# Autodesk Inventor assembly: ELEV_000_FULLASMBLY
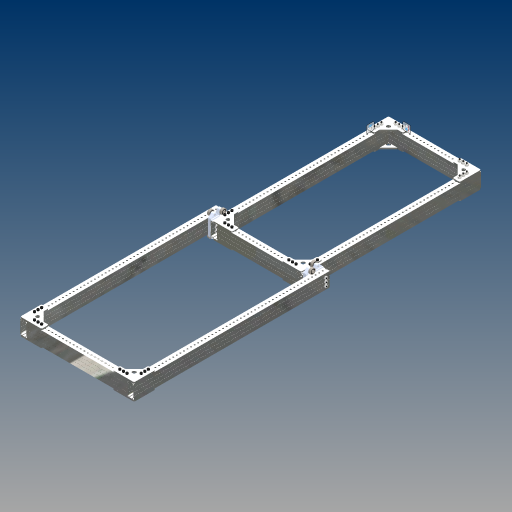
[picture p0: Inventor's stored thumbnail of the model, 512x512]
Saved by Autodesk Inventor 2024.3 (Build 283343000, 343)
## iProperties
Created: 2024-11-25
Part Number: ELEV_000_FULLASMBLY
Document SubType Name: Assembly
Designer: Kenji
Mass: 3407.89 g
Surface Area: 12378 cm^2
Volume: 1206.36 cm^3
Density: 2.82493 g/cm^3
Author: Kenji
## Documents named in this file (22)
- C:\Users\Kenji\Documents\GitHub\1622-2024-Casino-Clash-CAD-A-Thon\Elevator\ELEV_000_FULLASMBLY.iam
- C:\Users\Kenji\Documents\GitHub\1622-2024-Casino-Clash-CAD-A-Thon\Elevator\ELEV_001_BAR1(27.500 in).ipt
- C:\Users\Kenji\Documents\GitHub\1622-2024-Casino-Clash-CAD-A-Thon\Elevator\ELEV_002_BAR2(14.000 in).ipt
- C:\Users\Kenji\Documents\GitHub\1622-2024-Casino-Clash-CAD-A-Thon\Elevator\ELEV_003_BAR3(25.000 in).ipt
- C:\Users\Kenji\Documents\GitHub\1622-2024-Casino-Clash-CAD-A-Thon\COTS Library\Motion\BearingBlocks\ElevatorBlocks\WCP-0897_InlineBearingBlock.iam
- C:\Users\Kenji\Documents\GitHub\1622-2024-Casino-Clash-CAD-A-Thon\Elevator\ELEV_004_BAR4(12.000 in).ipt
- C:\Users\Kenji\Documents\GitHub\1622-2024-Casino-Clash-CAD-A-Thon\Elevator\ELEV_005_SUPBRK1.ipt
- C:\Users\Kenji\Documents\GitHub\1622-2024-Casino-Clash-CAD-A-Thon\COTS Library\Fasteners\Nuts\COTS_90633A411_Low-Strength Steel Thin Nylon-Insert Locknut_10-32.ipt
- C:\Users\Kenji\Documents\GitHub\1622-2024-Casino-Clash-CAD-A-Thon\Elevator\ELEV_006_SUPBRK1_THRD.ipt
- C:\Users\Kenji\Documents\GitHub\1622-2024-Casino-Clash-CAD-A-Thon\COTS Library\Fasteners\Bolts\Socket-Head\10-32\COTS_90044A121_Black-Oxide Alloy Steel Socket Head Screw_10-32_2.5in.ipt
- C:\Users\Kenji\Documents\GitHub\1622-2024-Casino-Clash-CAD-A-Thon\COTS Library\Fasteners\Bolts\Socket-Head\10-32\COTS_90044A202_Black-Oxide Alloy Steel Socket Head Screw_1-.375.ipt
- C:\Users\Kenji\Documents\GitHub\1622-2024-Casino-Clash-CAD-A-Thon\COTS Library\Fasteners\Bolts\Socket-Head\10-32\COTS_91251A342_Black-Oxide Alloy Steel Socket Head Screw_.5in.ipt
- C:\Users\Kenji\Documents\GitHub\1622-2024-Casino-Clash-CAD-A-Thon\Elevator\ELEV_007_SUPBRK2.ipt
- C:\Users\Kenji\Documents\GitHub\1622-2024-Casino-Clash-CAD-A-Thon\COTS Library\Fasteners\Bolts\Socket-Head\10-32\COTS_91251A359_Black-Oxide Alloy Steel Socket Head Screw_10-32_2_3-4in.ipt
- C:\Users\Kenji\Documents\GitHub\1622-2024-Casino-Clash-CAD-A-Thon\COTS Library\Fasteners\Nuts\COTS_90631A411_Low-Strength Steel Nylon-Insert Locknut_10-32.ipt
- C:\Users\Kenji\Documents\GitHub\1622-2024-Casino-Clash-CAD-A-Thon\Elevator\ELEV_008_SUPBRK3.ipt
- C:\Users\Kenji\Documents\GitHub\1622-2024-Casino-Clash-CAD-A-Thon\Elevator\ELEV_000_FULLASMBLY\AIP\FEA\ew6g7bhkw.fins
- C:\Users\Kenji\Documents\GitHub\1622-2024-Casino-Clash-CAD-A-Thon\Elevator\ELEV_000_FULLASMBLY\AIP\FEA\ew6g7bhkw.fsat
- C:\Users\Kenji\Documents\GitHub\1622-2024-Casino-Clash-CAD-A-Thon\Elevator\ELEV_000_FULLASMBLY\AIP\FEA\ew6g7bhkw.ftes
- C:\Users\Kenji\Documents\GitHub\1622-2024-Casino-Clash-CAD-A-Thon\Elevator\ELEV_000_FULLASMBLY\AIP\FEA\ew6g7bhkw.fwiz
- C:\Users\Kenji\Documents\GitHub\1622-2024-Casino-Clash-CAD-A-Thon\Elevator\ELEV_000_FULLASMBLY\AIP\FEA\ew6g7biao.fmsh
- C:\Users\Kenji\Documents\GitHub\1622-2024-Casino-Clash-CAD-A-Thon\Elevator\ELEV_000_FULLASMBLY\AIP\FEA\ew6g7bibk.fres
## Components (107 placed, 15 different names)
1. ELEV_001_BAR1(27.500 in):1 — Flush:1, Flush:2, Mate:1, Mate:2, Flush:7, Tangent:2, Mate:10, Flush:11, Mate:11, Mate:78, Mate:133, Mate:136, Mate:137
2. ELEV_001_BAR1(27.500 in):2 — Flush:1, Flush:2, Mate:1, Flush:3, Flush:4, Mate:3, Angle:1, Mate:4, Flush:8, Angle:2, Mate:74, Mate:128, Mate:131
3. ELEV_002_BAR2(14.000 in):1 — Flush:3, Flush:4, Mate:2, Mate:127, Flush:24, Mate:132, Mate:134, Mate:135
4. ELEV_003_BAR3(25.000 in):1 — Flush:5, Flush:6, Flush:7, Mate:8, Flush:10, Mate:9, Mate:82, Flush:19, Flush:21
5. ELEV_003_BAR3(25.000 in):2 — Flush:5, Flush:6, Tangent:1, Angle:2, Mate:5, Angle:3, Mate:6, Flush:9, Mate:12, Flush:12, Flush:13, Mate:13, Flush:14, Mate:14, Mate:16, Mate:62, Mate:86, Flush:17, Flush:22
6. WCP-0897_InlineBearingBlock:1 [sub-assembly] — Mate:5, Angle:3, Mate:6, Flush:9, Mate:83, Mate:84
7. WCP-0897_InlineBearingBlock:2 [sub-assembly] — Mate:3, Angle:1, Mate:4, Tangent:1, Flush:8, Mate:71, Mate:72
8. WCP-0897_InlineBearingBlock:3 [sub-assembly] — Mate:8, Flush:10, Mate:9, Tangent:2, Mate:37, Mate:79, Mate:80
9. WCP-0897_InlineBearingBlock:4 [sub-assembly] — Mate:10, Flush:11, Mate:11, Mate:37, Mate:75, Mate:76
10. ELEV_004_BAR4(12.000 in):1 — Mate:12, Flush:12, Flush:13, Mate:17, Mate:18, Mate:19, Angle:4, Mate:20, Mate:42, Mate:45, Mate:60, Flush:15, Mate:61
11. ELEV_004_BAR4(12.000 in):2 — Mate:13, Flush:14, Mate:14, Flush:16, Flush:18, Mate:88, Flush:20, Mate:89, Flush:23, Mate:90, Mate:110
12. ELEV_005_SUPBRK1:1 — Mate:16, Mate:17, Mate:18, Mate:67, Mate:68, Mate:69, Mate:70
13. ELEV_005_SUPBRK1:2 — Mate:19, Angle:4, Mate:20, Mate:63, Mate:64, Mate:65, Mate:66
14. ELEV_006_SUPBRK1_THRD:1 — Mate:42, Mate:61, Mate:62
15. ELEV_006_SUPBRK1_THRD:2 — Mate:45, Mate:60, Flush:15
16. ELEV_007_SUPBRK2:1 — Flush:16, Flush:17, Mate:110, Mate:120, Mate:122
17. ELEV_007_SUPBRK2:2 — Flush:18, Flush:19, Mate:88, Mate:124, Mate:126
18. ELEV_007_SUPBRK2:3 — Flush:22, Flush:23, Mate:90, Mate:115, Mate:116, Mate:117, Mate:118
19. ELEV_007_SUPBRK2:4 — Flush:20, Flush:21, Mate:89, Mate:111, Mate:112, Mate:113, Mate:114
20. ELEV_008_SUPBRK3:1 — Mate:127, Flush:24, Mate:128, Mate:129, Mate:130, Mate:138, Mate:139, Mate:144, Mate:145
21. ELEV_008_SUPBRK3:2 — Mate:129, Mate:130, Mate:131, Mate:148, Mate:149
22. ELEV_008_SUPBRK3:3 — Mate:132, Mate:133, Mate:134, Mate:151, Mate:153
23. ELEV_008_SUPBRK3:4 — Mate:135, Mate:136, Mate:137, Mate:140, Mate:141, Mate:142, Mate:143
24. COTS_90044A121_Black-Oxide Alloy Steel Socket Head Screw_10-32_2.5in:1 — Mate:63, Mate:64
25. COTS_90044A121_Black-Oxide Alloy Steel Socket Head Screw_10-32_2.5in:5
26. COTS_90044A121_Black-Oxide Alloy Steel Socket Head Screw_10-32_2.5in:6
27. COTS_90044A121_Black-Oxide Alloy Steel Socket Head Screw_10-32_2.5in:4 — Mate:65, Mate:66
28. COTS_90044A121_Black-Oxide Alloy Steel Socket Head Screw_10-32_2.5in:7
29. COTS_90044A121_Black-Oxide Alloy Steel Socket Head Screw_10-32_2.5in:8
30. COTS_90044A121_Black-Oxide Alloy Steel Socket Head Screw_10-32_2.5in:3 — Mate:68, Mate:70
31. COTS_90044A121_Black-Oxide Alloy Steel Socket Head Screw_10-32_2.5in:9
32. COTS_90044A121_Black-Oxide Alloy Steel Socket Head Screw_10-32_2.5in:10
33. COTS_90044A121_Black-Oxide Alloy Steel Socket Head Screw_10-32_2.5in:2 — Mate:67, Mate:69
34. COTS_90044A121_Black-Oxide Alloy Steel Socket Head Screw_10-32_2.5in:11
35. COTS_90044A121_Black-Oxide Alloy Steel Socket Head Screw_10-32_2.5in:12
36. COTS_90044A202_Black-Oxide Alloy Steel Socket Head Screw_1-.375:1 — Mate:71, Mate:72, Mate:73
37. COTS_90633A411_Low-Strength Steel Thin Nylon-Insert Locknut_10-32:1 — Mate:73, Mate:74
38. COTS_90044A202_Black-Oxide Alloy Steel Socket Head Screw_1-.375:2
39. COTS_90633A411_Low-Strength Steel Thin Nylon-Insert Locknut_10-32:2
40. COTS_90044A202_Black-Oxide Alloy Steel Socket Head Screw_1-.375:3
41. COTS_90633A411_Low-Strength Steel Thin Nylon-Insert Locknut_10-32:3
42. COTS_90633A411_Low-Strength Steel Thin Nylon-Insert Locknut_10-32:4 — Mate:77, Mate:78
43. COTS_90044A202_Black-Oxide Alloy Steel Socket Head Screw_1-.375:4 — Mate:75, Mate:76, Mate:77
44. COTS_90633A411_Low-Strength Steel Thin Nylon-Insert Locknut_10-32:5
45. COTS_90044A202_Black-Oxide Alloy Steel Socket Head Screw_1-.375:5
46. COTS_90633A411_Low-Strength Steel Thin Nylon-Insert Locknut_10-32:6
47. COTS_90044A202_Black-Oxide Alloy Steel Socket Head Screw_1-.375:6
48. COTS_91251A342_Black-Oxide Alloy Steel Socket Head Screw_.5in:1 — Mate:79, Mate:80, Mate:81
49. COTS_90633A411_Low-Strength Steel Thin Nylon-Insert Locknut_10-32:7 — Mate:81, Mate:82
50. COTS_91251A342_Black-Oxide Alloy Steel Socket Head Screw_.5in:2
51. COTS_90633A411_Low-Strength Steel Thin Nylon-Insert Locknut_10-32:8
52. COTS_91251A342_Black-Oxide Alloy Steel Socket Head Screw_.5in:3
53. COTS_90633A411_Low-Strength Steel Thin Nylon-Insert Locknut_10-32:9
54. COTS_90633A411_Low-Strength Steel Thin Nylon-Insert Locknut_10-32:10 — Mate:85, Mate:86
55. COTS_91251A342_Black-Oxide Alloy Steel Socket Head Screw_.5in:4 — Mate:83, Mate:84, Mate:85
56. COTS_90633A411_Low-Strength Steel Thin Nylon-Insert Locknut_10-32:11
57. COTS_91251A342_Black-Oxide Alloy Steel Socket Head Screw_.5in:5
58. COTS_90633A411_Low-Strength Steel Thin Nylon-Insert Locknut_10-32:12
59. COTS_91251A342_Black-Oxide Alloy Steel Socket Head Screw_.5in:6
60. COTS_91251A359_Black-Oxide Alloy Steel Socket Head Screw_10-32_2_3-4in:3 — Mate:111, Mate:112, Mate:123
61. COTS_90631A411_Low-Strength Steel Nylon-Insert Locknut_10-32:2 — Mate:123, Mate:124
62. COTS_91251A359_Black-Oxide Alloy Steel Socket Head Screw_10-32_2_3-4in:5
63. COTS_90631A411_Low-Strength Steel Nylon-Insert Locknut_10-32:5
64. COTS_91251A359_Black-Oxide Alloy Steel Socket Head Screw_10-32_2_3-4in:6
65. COTS_90631A411_Low-Strength Steel Nylon-Insert Locknut_10-32:6
66. COTS_91251A359_Black-Oxide Alloy Steel Socket Head Screw_10-32_2_3-4in:1 — Mate:113, Mate:114, Mate:125
67. COTS_91251A359_Black-Oxide Alloy Steel Socket Head Screw_10-32_2_3-4in:7
68. COTS_91251A359_Black-Oxide Alloy Steel Socket Head Screw_10-32_2_3-4in:8
69. COTS_91251A359_Black-Oxide Alloy Steel Socket Head Screw_10-32_2_3-4in:2 — Mate:115, Mate:118, Mate:121
70. COTS_90631A411_Low-Strength Steel Nylon-Insert Locknut_10-32:4 — Mate:121, Mate:122
71. COTS_91251A359_Black-Oxide Alloy Steel Socket Head Screw_10-32_2_3-4in:9
72. COTS_90631A411_Low-Strength Steel Nylon-Insert Locknut_10-32:7
73. COTS_91251A359_Black-Oxide Alloy Steel Socket Head Screw_10-32_2_3-4in:10
74. COTS_90631A411_Low-Strength Steel Nylon-Insert Locknut_10-32:8
75. COTS_90631A411_Low-Strength Steel Nylon-Insert Locknut_10-32:3 — Mate:119, Mate:120
76. COTS_91251A359_Black-Oxide Alloy Steel Socket Head Screw_10-32_2_3-4in:4 — Mate:116, Mate:117, Mate:119
77. COTS_90631A411_Low-Strength Steel Nylon-Insert Locknut_10-32:9
78. COTS_91251A359_Black-Oxide Alloy Steel Socket Head Screw_10-32_2_3-4in:11
79. COTS_90631A411_Low-Strength Steel Nylon-Insert Locknut_10-32:10
80. COTS_91251A359_Black-Oxide Alloy Steel Socket Head Screw_10-32_2_3-4in:12
81. COTS_90631A411_Low-Strength Steel Nylon-Insert Locknut_10-32:1 — Mate:125, Mate:126
82. COTS_90631A411_Low-Strength Steel Nylon-Insert Locknut_10-32:11
83. COTS_90631A411_Low-Strength Steel Nylon-Insert Locknut_10-32:12
84. COTS_90631A411_Low-Strength Steel Nylon-Insert Locknut_10-32:14 — Mate:152, Mate:153
85. COTS_91251A359_Black-Oxide Alloy Steel Socket Head Screw_10-32_2_3-4in:14 — Mate:140, Mate:143, Mate:152
86. COTS_90631A411_Low-Strength Steel Nylon-Insert Locknut_10-32:17
87. COTS_91251A359_Black-Oxide Alloy Steel Socket Head Screw_10-32_2_3-4in:17
88. COTS_90631A411_Low-Strength Steel Nylon-Insert Locknut_10-32:18
89. COTS_91251A359_Black-Oxide Alloy Steel Socket Head Screw_10-32_2_3-4in:18
90. COTS_91251A359_Black-Oxide Alloy Steel Socket Head Screw_10-32_2_3-4in:13 — Mate:141, Mate:142, Mate:150
91. COTS_90631A411_Low-Strength Steel Nylon-Insert Locknut_10-32:15 — Mate:150, Mate:151
92. COTS_91251A359_Black-Oxide Alloy Steel Socket Head Screw_10-32_2_3-4in:19
93. COTS_90631A411_Low-Strength Steel Nylon-Insert Locknut_10-32:19
94. COTS_91251A359_Black-Oxide Alloy Steel Socket Head Screw_10-32_2_3-4in:20
95. COTS_90631A411_Low-Strength Steel Nylon-Insert Locknut_10-32:20
96. COTS_91251A359_Black-Oxide Alloy Steel Socket Head Screw_10-32_2_3-4in:15 — Mate:139, Mate:145, Mate:147
97. COTS_90631A411_Low-Strength Steel Nylon-Insert Locknut_10-32:13 — Mate:147, Mate:149
98. COTS_91251A359_Black-Oxide Alloy Steel Socket Head Screw_10-32_2_3-4in:21
99. COTS_90631A411_Low-Strength Steel Nylon-Insert Locknut_10-32:21
100. COTS_91251A359_Black-Oxide Alloy Steel Socket Head Screw_10-32_2_3-4in:22
101. COTS_90631A411_Low-Strength Steel Nylon-Insert Locknut_10-32:22
102. COTS_90631A411_Low-Strength Steel Nylon-Insert Locknut_10-32:16 — Mate:146, Mate:148
103. COTS_91251A359_Black-Oxide Alloy Steel Socket Head Screw_10-32_2_3-4in:16 — Mate:138, Mate:144, Mate:146
104. COTS_90631A411_Low-Strength Steel Nylon-Insert Locknut_10-32:23
105. COTS_91251A359_Black-Oxide Alloy Steel Socket Head Screw_10-32_2_3-4in:23
106. COTS_90631A411_Low-Strength Steel Nylon-Insert Locknut_10-32:24
107. COTS_91251A359_Black-Oxide Alloy Steel Socket Head Screw_10-32_2_3-4in:24
## Component patterns: (3 elements, first: COTS_90044A121_Black-Oxide Alloy Steel Socket Head Screw_10-32_2.5in:1), (3 elements, first: COTS_90044A121_Black-Oxide Alloy Steel Socket Head Screw_10-32_2.5in:4), (3 elements, first: COTS_90044A121_Black-Oxide Alloy Steel Socket Head Screw_10-32_2.5in:3), (3 elements, first: COTS_90044A121_Black-Oxide Alloy Steel Socket Head Screw_10-32_2.5in:2), (3 elements, first: COTS_90044A202_Black-Oxide Alloy Steel Socket Head Screw_1-.375:1 + COTS_90633A411_Low-Strength Steel Thin Nylon-Insert Locknut_10-32:1), (3 elements, first: COTS_90633A411_Low-Strength Steel Thin Nylon-Insert Locknut_10-32:4 + COTS_90044A202_Black-Oxide Alloy Steel Socket Head Screw_1-.375:4), (3 elements, first: COTS_91251A342_Black-Oxide Alloy Steel Socket Head Screw_.5in:1 + COTS_90633A411_Low-Strength Steel Thin Nylon-Insert Locknut_10-32:7), (3 elements, first: COTS_90633A411_Low-Strength Steel Thin Nylon-Insert Locknut_10-32:10 + COTS_91251A342_Black-Oxide Alloy Steel Socket Head Screw_.5in:4), (3 elements, first: COTS_91251A359_Black-Oxide Alloy Steel Socket Head Screw_10-32_2_3-4in:3 + COTS_90631A411_Low-Strength Steel Nylon-Insert Locknut_10-32:2), (3 elements, first: COTS_91251A359_Black-Oxide Alloy Steel Socket Head Screw_10-32_2_3-4in:1), (3 elements, first: COTS_91251A359_Black-Oxide Alloy Steel Socket Head Screw_10-32_2_3-4in:2 + COTS_90631A411_Low-Strength Steel Nylon-Insert Locknut_10-32:4), (3 elements, first: COTS_90631A411_Low-Strength Steel Nylon-Insert Locknut_10-32:3 + COTS_91251A359_Black-Oxide Alloy Steel Socket Head Screw_10-32_2_3-4in:4), (3 elements, first: COTS_90631A411_Low-Strength Steel Nylon-Insert Locknut_10-32:1), (3 elements, first: COTS_90631A411_Low-Strength Steel Nylon-Insert Locknut_10-32:14 + COTS_91251A359_Black-Oxide Alloy Steel Socket Head Screw_10-32_2_3-4in:14), (3 elements, first: COTS_91251A359_Black-Oxide Alloy Steel Socket Head Screw_10-32_2_3-4in:13 + COTS_90631A411_Low-Strength Steel Nylon-Insert Locknut_10-32:15), (3 elements, first: COTS_91251A359_Black-Oxide Alloy Steel Socket Head Screw_10-32_2_3-4in:15 + COTS_90631A411_Low-Strength Steel Nylon-Insert Locknut_10-32:13), (3 elements, first: COTS_90631A411_Low-Strength Steel Nylon-Insert Locknut_10-32:16 + COTS_91251A359_Black-Oxide Alloy Steel Socket Head Screw_10-32_2_3-4in:16)
## Relationships (125: Mate 95, Flush 24, Angle 4, Tangent 2)
- Flush:1: ELEV_001_BAR1(27.500 in):1 ↔ ELEV_001_BAR1(27.500 in):2
- Flush:2: ELEV_001_BAR1(27.500 in):1 ↔ ELEV_001_BAR1(27.500 in):2
- Mate:1 (355.6 mm): ELEV_001_BAR1(27.500 in):1 ↔ ELEV_001_BAR1(27.500 in):2
- Flush:3: ELEV_001_BAR1(27.500 in):2 ↔ ELEV_002_BAR2(14.000 in):1
- Flush:4: ELEV_001_BAR1(27.500 in):2 ↔ ELEV_002_BAR2(14.000 in):1
- Mate:2: ELEV_001_BAR1(27.500 in):1 ↔ ELEV_002_BAR2(14.000 in):1
- Flush:5: ELEV_003_BAR3(25.000 in):1 ↔ ELEV_003_BAR3(25.000 in):2
- Flush:6: ELEV_003_BAR3(25.000 in):1 ↔ ELEV_003_BAR3(25.000 in):2
- Flush:7: ELEV_001_BAR1(27.500 in):1 ↔ ELEV_003_BAR3(25.000 in):1
- Mate:3: ELEV_001_BAR1(27.500 in):2 ↔ WCP-0897_InlineBearingBlock:2
- Angle:1 (0 deg): ELEV_001_BAR1(27.500 in):2 ↔ WCP-0897_InlineBearingBlock:2
- Mate:4: ELEV_001_BAR1(27.500 in):2 ↔ WCP-0897_InlineBearingBlock:2
- Tangent:1: ELEV_003_BAR3(25.000 in):2 ↔ WCP-0897_InlineBearingBlock:2
- Flush:8: ELEV_001_BAR1(27.500 in):2 ↔ WCP-0897_InlineBearingBlock:2
- Angle:2 (0 deg): ELEV_001_BAR1(27.500 in):2 ↔ ELEV_003_BAR3(25.000 in):2
- Mate:5: ELEV_003_BAR3(25.000 in):2 ↔ WCP-0897_InlineBearingBlock:1
- Angle:3 (0 deg): ELEV_003_BAR3(25.000 in):2 ↔ WCP-0897_InlineBearingBlock:1
- Mate:6: ELEV_003_BAR3(25.000 in):2 ↔ WCP-0897_InlineBearingBlock:1
- Flush:9: ELEV_003_BAR3(25.000 in):2 ↔ WCP-0897_InlineBearingBlock:1
- Mate:8: ELEV_003_BAR3(25.000 in):1 ↔ WCP-0897_InlineBearingBlock:3
- Flush:10: ELEV_003_BAR3(25.000 in):1 ↔ WCP-0897_InlineBearingBlock:3
- Mate:9: ELEV_003_BAR3(25.000 in):1 ↔ WCP-0897_InlineBearingBlock:3
- Tangent:2: ELEV_001_BAR1(27.500 in):1 ↔ WCP-0897_InlineBearingBlock:3
- Mate:10: ELEV_001_BAR1(27.500 in):1 ↔ WCP-0897_InlineBearingBlock:4
- Flush:11: ELEV_001_BAR1(27.500 in):1 ↔ WCP-0897_InlineBearingBlock:4
- Mate:11: ELEV_001_BAR1(27.500 in):1 ↔ WCP-0897_InlineBearingBlock:4
- Mate:12: ELEV_003_BAR3(25.000 in):2 ↔ ELEV_004_BAR4(12.000 in):1
- Flush:12: ELEV_003_BAR3(25.000 in):2 ↔ ELEV_004_BAR4(12.000 in):1
- Flush:13: ELEV_003_BAR3(25.000 in):2 ↔ ELEV_004_BAR4(12.000 in):1
- Mate:13: ELEV_003_BAR3(25.000 in):2 ↔ ELEV_004_BAR4(12.000 in):2
- Flush:14: ELEV_003_BAR3(25.000 in):2 ↔ ELEV_004_BAR4(12.000 in):2
- Mate:14: ELEV_003_BAR3(25.000 in):2 ↔ ELEV_004_BAR4(12.000 in):2
- Mate:16: ELEV_003_BAR3(25.000 in):2 ↔ ELEV_005_SUPBRK1:1
- Mate:17: ELEV_004_BAR4(12.000 in):1 ↔ ELEV_005_SUPBRK1:1
- Mate:18: ELEV_004_BAR4(12.000 in):1 ↔ ELEV_005_SUPBRK1:1
- Mate:19: ELEV_004_BAR4(12.000 in):1 ↔ ELEV_005_SUPBRK1:2
- Angle:4 (0 deg): ELEV_004_BAR4(12.000 in):1 ↔ ELEV_005_SUPBRK1:2
- Mate:20: ELEV_004_BAR4(12.000 in):1 ↔ ELEV_005_SUPBRK1:2
- Mate:37: WCP-0897_InlineBearingBlock:3 ↔ WCP-0897_InlineBearingBlock:4
- Mate:42: ELEV_004_BAR4(12.000 in):1 ↔ ELEV_006_SUPBRK1_THRD:1
- Mate:45: ELEV_004_BAR4(12.000 in):1 ↔ ELEV_006_SUPBRK1_THRD:2
- Mate:60: ELEV_004_BAR4(12.000 in):1 ↔ ELEV_006_SUPBRK1_THRD:2
- Flush:15: ELEV_004_BAR4(12.000 in):1 ↔ ELEV_006_SUPBRK1_THRD:2
- Mate:61: ELEV_004_BAR4(12.000 in):1 ↔ ELEV_006_SUPBRK1_THRD:1
- Mate:62: ELEV_003_BAR3(25.000 in):2 ↔ ELEV_006_SUPBRK1_THRD:1
- Mate:63: ELEV_005_SUPBRK1:2 ↔ COTS_90044A121_Black-Oxide Alloy Steel Socket Head Screw_10-32_2.5in:1
- Mate:64: ELEV_005_SUPBRK1:2 ↔ COTS_90044A121_Black-Oxide Alloy Steel Socket Head Screw_10-32_2.5in:1
- Mate:65: ELEV_005_SUPBRK1:2 ↔ COTS_90044A121_Black-Oxide Alloy Steel Socket Head Screw_10-32_2.5in:4
- Mate:66: ELEV_005_SUPBRK1:2 ↔ COTS_90044A121_Black-Oxide Alloy Steel Socket Head Screw_10-32_2.5in:4
- Mate:67: ELEV_005_SUPBRK1:1 ↔ COTS_90044A121_Black-Oxide Alloy Steel Socket Head Screw_10-32_2.5in:2
- Mate:68: ELEV_005_SUPBRK1:1 ↔ COTS_90044A121_Black-Oxide Alloy Steel Socket Head Screw_10-32_2.5in:3
- Mate:69: ELEV_005_SUPBRK1:1 ↔ COTS_90044A121_Black-Oxide Alloy Steel Socket Head Screw_10-32_2.5in:2
- Mate:70: ELEV_005_SUPBRK1:1 ↔ COTS_90044A121_Black-Oxide Alloy Steel Socket Head Screw_10-32_2.5in:3
- Mate:71: WCP-0897_InlineBearingBlock:2 ↔ COTS_90044A202_Black-Oxide Alloy Steel Socket Head Screw_1-.375:1
- Mate:72: WCP-0897_InlineBearingBlock:2 ↔ COTS_90044A202_Black-Oxide Alloy Steel Socket Head Screw_1-.375:1
- Mate:73: COTS_90044A202_Black-Oxide Alloy Steel Socket Head Screw_1-.375:1 ↔ COTS_90633A411_Low-Strength Steel Thin Nylon-Insert Locknut_10-32:1
- Mate:74: ELEV_001_BAR1(27.500 in):2 ↔ COTS_90633A411_Low-Strength Steel Thin Nylon-Insert Locknut_10-32:1
- Mate:75: WCP-0897_InlineBearingBlock:4 ↔ COTS_90044A202_Black-Oxide Alloy Steel Socket Head Screw_1-.375:4
- Mate:76: WCP-0897_InlineBearingBlock:4 ↔ COTS_90044A202_Black-Oxide Alloy Steel Socket Head Screw_1-.375:4
- Mate:77: COTS_90633A411_Low-Strength Steel Thin Nylon-Insert Locknut_10-32:4 ↔ COTS_90044A202_Black-Oxide Alloy Steel Socket Head Screw_1-.375:4
- Mate:78: ELEV_001_BAR1(27.500 in):1 ↔ COTS_90633A411_Low-Strength Steel Thin Nylon-Insert Locknut_10-32:4
- Mate:79: WCP-0897_InlineBearingBlock:3 ↔ COTS_91251A342_Black-Oxide Alloy Steel Socket Head Screw_.5in:1
- Mate:80: WCP-0897_InlineBearingBlock:3 ↔ COTS_91251A342_Black-Oxide Alloy Steel Socket Head Screw_.5in:1
- Mate:81: COTS_91251A342_Black-Oxide Alloy Steel Socket Head Screw_.5in:1 ↔ COTS_90633A411_Low-Strength Steel Thin Nylon-Insert Locknut_10-32:7
- Mate:82: ELEV_003_BAR3(25.000 in):1 ↔ COTS_90633A411_Low-Strength Steel Thin Nylon-Insert Locknut_10-32:7
- Mate:83: WCP-0897_InlineBearingBlock:1 ↔ COTS_91251A342_Black-Oxide Alloy Steel Socket Head Screw_.5in:4
- Mate:84: WCP-0897_InlineBearingBlock:1 ↔ COTS_91251A342_Black-Oxide Alloy Steel Socket Head Screw_.5in:4
- Mate:85: COTS_90633A411_Low-Strength Steel Thin Nylon-Insert Locknut_10-32:10 ↔ COTS_91251A342_Black-Oxide Alloy Steel Socket Head Screw_.5in:4
- Mate:86: ELEV_003_BAR3(25.000 in):2 ↔ COTS_90633A411_Low-Strength Steel Thin Nylon-Insert Locknut_10-32:10
- Flush:16: ELEV_004_BAR4(12.000 in):2 ↔ ELEV_007_SUPBRK2:1
- Flush:17: ELEV_003_BAR3(25.000 in):2 ↔ ELEV_007_SUPBRK2:1
- Flush:18: ELEV_004_BAR4(12.000 in):2 ↔ ELEV_007_SUPBRK2:2
- Flush:19: ELEV_003_BAR3(25.000 in):1 ↔ ELEV_007_SUPBRK2:2
- Mate:88: ELEV_004_BAR4(12.000 in):2 ↔ ELEV_007_SUPBRK2:2
- Flush:20: ELEV_004_BAR4(12.000 in):2 ↔ ELEV_007_SUPBRK2:4
- Flush:21: ELEV_003_BAR3(25.000 in):1 ↔ ELEV_007_SUPBRK2:4
- Mate:89: ELEV_004_BAR4(12.000 in):2 ↔ ELEV_007_SUPBRK2:4
- Flush:22: ELEV_003_BAR3(25.000 in):2 ↔ ELEV_007_SUPBRK2:3
- Flush:23: ELEV_004_BAR4(12.000 in):2 ↔ ELEV_007_SUPBRK2:3
- Mate:90: ELEV_004_BAR4(12.000 in):2 ↔ ELEV_007_SUPBRK2:3
- Mate:110: ELEV_004_BAR4(12.000 in):2 ↔ ELEV_007_SUPBRK2:1
- Mate:111: ELEV_007_SUPBRK2:4 ↔ COTS_91251A359_Black-Oxide Alloy Steel Socket Head Screw_10-32_2_3-4in:3
- Mate:112: ELEV_007_SUPBRK2:4 ↔ COTS_91251A359_Black-Oxide Alloy Steel Socket Head Screw_10-32_2_3-4in:3
- Mate:113: ELEV_007_SUPBRK2:4 ↔ COTS_91251A359_Black-Oxide Alloy Steel Socket Head Screw_10-32_2_3-4in:1
- Mate:114: ELEV_007_SUPBRK2:4 ↔ COTS_91251A359_Black-Oxide Alloy Steel Socket Head Screw_10-32_2_3-4in:1
- Mate:115: ELEV_007_SUPBRK2:3 ↔ COTS_91251A359_Black-Oxide Alloy Steel Socket Head Screw_10-32_2_3-4in:2
- Mate:116: ELEV_007_SUPBRK2:3 ↔ COTS_91251A359_Black-Oxide Alloy Steel Socket Head Screw_10-32_2_3-4in:4
- Mate:117: ELEV_007_SUPBRK2:3 ↔ COTS_91251A359_Black-Oxide Alloy Steel Socket Head Screw_10-32_2_3-4in:4
- Mate:118: ELEV_007_SUPBRK2:3 ↔ COTS_91251A359_Black-Oxide Alloy Steel Socket Head Screw_10-32_2_3-4in:2
- Mate:119: COTS_90631A411_Low-Strength Steel Nylon-Insert Locknut_10-32:3 ↔ COTS_91251A359_Black-Oxide Alloy Steel Socket Head Screw_10-32_2_3-4in:4
- Mate:120: ELEV_007_SUPBRK2:1 ↔ COTS_90631A411_Low-Strength Steel Nylon-Insert Locknut_10-32:3
- Mate:121: COTS_91251A359_Black-Oxide Alloy Steel Socket Head Screw_10-32_2_3-4in:2 ↔ COTS_90631A411_Low-Strength Steel Nylon-Insert Locknut_10-32:4
- Mate:122: ELEV_007_SUPBRK2:1 ↔ COTS_90631A411_Low-Strength Steel Nylon-Insert Locknut_10-32:4
- Mate:123: COTS_91251A359_Black-Oxide Alloy Steel Socket Head Screw_10-32_2_3-4in:3 ↔ COTS_90631A411_Low-Strength Steel Nylon-Insert Locknut_10-32:2
- Mate:124: ELEV_007_SUPBRK2:2 ↔ COTS_90631A411_Low-Strength Steel Nylon-Insert Locknut_10-32:2
- Mate:125: COTS_91251A359_Black-Oxide Alloy Steel Socket Head Screw_10-32_2_3-4in:1 ↔ COTS_90631A411_Low-Strength Steel Nylon-Insert Locknut_10-32:1
- Mate:126: ELEV_007_SUPBRK2:2 ↔ COTS_90631A411_Low-Strength Steel Nylon-Insert Locknut_10-32:1
- Mate:127: ELEV_002_BAR2(14.000 in):1 ↔ ELEV_008_SUPBRK3:1
- Flush:24: ELEV_002_BAR2(14.000 in):1 ↔ ELEV_008_SUPBRK3:1
- Mate:128: ELEV_001_BAR1(27.500 in):2 ↔ ELEV_008_SUPBRK3:1
- Mate:129: ELEV_008_SUPBRK3:1 ↔ ELEV_008_SUPBRK3:2
- Mate:130: ELEV_008_SUPBRK3:1 ↔ ELEV_008_SUPBRK3:2
- Mate:131: ELEV_001_BAR1(27.500 in):2 ↔ ELEV_008_SUPBRK3:2
- Mate:132: ELEV_002_BAR2(14.000 in):1 ↔ ELEV_008_SUPBRK3:3
- Mate:133: ELEV_001_BAR1(27.500 in):1 ↔ ELEV_008_SUPBRK3:3
- Mate:134: ELEV_002_BAR2(14.000 in):1 ↔ ELEV_008_SUPBRK3:3
- Mate:135: ELEV_002_BAR2(14.000 in):1 ↔ ELEV_008_SUPBRK3:4
- Mate:136: ELEV_001_BAR1(27.500 in):1 ↔ ELEV_008_SUPBRK3:4
- Mate:137: ELEV_001_BAR1(27.500 in):1 ↔ ELEV_008_SUPBRK3:4
- Mate:138: ELEV_008_SUPBRK3:1 ↔ COTS_91251A359_Black-Oxide Alloy Steel Socket Head Screw_10-32_2_3-4in:16
- Mate:139: ELEV_008_SUPBRK3:1 ↔ COTS_91251A359_Black-Oxide Alloy Steel Socket Head Screw_10-32_2_3-4in:15
- Mate:140: ELEV_008_SUPBRK3:4 ↔ COTS_91251A359_Black-Oxide Alloy Steel Socket Head Screw_10-32_2_3-4in:14
- Mate:141: ELEV_008_SUPBRK3:4 ↔ COTS_91251A359_Black-Oxide Alloy Steel Socket Head Screw_10-32_2_3-4in:13
- Mate:142: ELEV_008_SUPBRK3:4 ↔ COTS_91251A359_Black-Oxide Alloy Steel Socket Head Screw_10-32_2_3-4in:13
- Mate:143: ELEV_008_SUPBRK3:4 ↔ COTS_91251A359_Black-Oxide Alloy Steel Socket Head Screw_10-32_2_3-4in:14
- Mate:144: ELEV_008_SUPBRK3:1 ↔ COTS_91251A359_Black-Oxide Alloy Steel Socket Head Screw_10-32_2_3-4in:16
- Mate:145: ELEV_008_SUPBRK3:1 ↔ COTS_91251A359_Black-Oxide Alloy Steel Socket Head Screw_10-32_2_3-4in:15
- Mate:146: COTS_90631A411_Low-Strength Steel Nylon-Insert Locknut_10-32:16 ↔ COTS_91251A359_Black-Oxide Alloy Steel Socket Head Screw_10-32_2_3-4in:16
- Mate:147: COTS_91251A359_Black-Oxide Alloy Steel Socket Head Screw_10-32_2_3-4in:15 ↔ COTS_90631A411_Low-Strength Steel Nylon-Insert Locknut_10-32:13
- Mate:148: ELEV_008_SUPBRK3:2 ↔ COTS_90631A411_Low-Strength Steel Nylon-Insert Locknut_10-32:16
- Mate:149: ELEV_008_SUPBRK3:2 ↔ COTS_90631A411_Low-Strength Steel Nylon-Insert Locknut_10-32:13
- Mate:150: COTS_91251A359_Black-Oxide Alloy Steel Socket Head Screw_10-32_2_3-4in:13 ↔ COTS_90631A411_Low-Strength Steel Nylon-Insert Locknut_10-32:15
- Mate:151: ELEV_008_SUPBRK3:3 ↔ COTS_90631A411_Low-Strength Steel Nylon-Insert Locknut_10-32:15
- Mate:152: COTS_90631A411_Low-Strength Steel Nylon-Insert Locknut_10-32:14 ↔ COTS_91251A359_Black-Oxide Alloy Steel Socket Head Screw_10-32_2_3-4in:14
- Mate:153: ELEV_008_SUPBRK3:3 ↔ COTS_90631A411_Low-Strength Steel Nylon-Insert Locknut_10-32:14
## Named parameters: sa_0 = 35585.8
note: some values were not read from the file. Shown as the stored number, unit unknown: "sa_0".
